# Autodesk Inventor assembly: The wheel
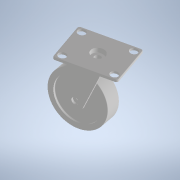
[picture p0: Inventor's stored thumbnail of the model, 180x180]
Saved by Autodesk Inventor 2022 (Build 260153000, 153)
## iProperties
Created: 2021-07-10
Part Number: The wheel
Document SubType Name: Assembly
Designer: fanam
Author: fanam
## Documents named in this file (4)
- C:\Users\fanam\Documents\The wheel.iam
- C:\Users\fanam\OneDrive\سطح المكتب\wheel part 1.ipt
- C:\Users\fanam\OneDrive\سطح المكتب\wheel part 2.ipt
- C:\Users\fanam\OneDrive\سطح المكتب\wheel part 3.ipt
## Components (3 placed, 3 different names)
1. wheel part 1:1 — Insert:2
2. wheel part 2:1 — Insert:1, Insert:2
3. wheel part 3:2 — Insert:1
## Relationships (2: Insert 2)
- Insert:1 (1 mm): wheel part 2:1 ↔ wheel part 3:2
- Insert:2: wheel part 1:1 ↔ wheel part 2:1
